# Autodesk Inventor assembly: Голень в сборе_MIR
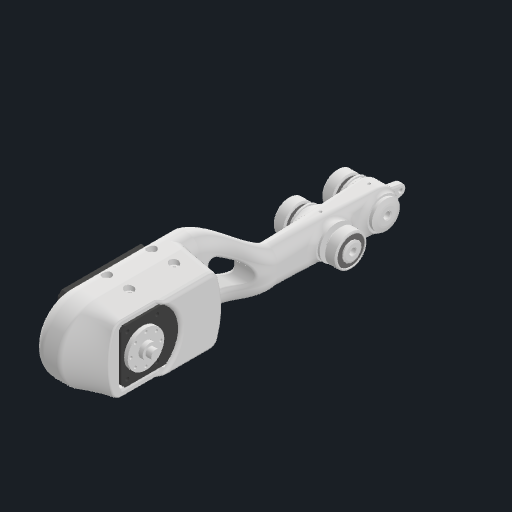
[picture p0: Inventor's stored thumbnail of the model, 512x512]
Saved by Autodesk Inventor 2025 (Build 290162010, 162A)
## iProperties
Created: 2024-12-05
Part Number: Голень в сборе_MIR
Document SubType Name: Assembly
Designer: Edward_Higgins
Author: Edward_Higgins
## Documents named in this file (8)
- D:\Users\Edward_Higgins\Desktop\ZAVOD\Робот Сколково\Голень в сборе_MIR.iam
- D:\Users\Edward_Higgins\Desktop\ZAVOD\Робот Сколково\DYNAMIXEL XM430-W350.ipt
- D:\Users\Edward_Higgins\Desktop\ZAVOD\Робот Сколково\Нога_MIR.ipt
- D:\Users\Edward_Higgins\Desktop\ZAVOD\Робот Сколково\Подшипник.ipt
- D:\Users\Edward_Higgins\Desktop\ZAVOD\Робот Сколково\Ось двусторонняя.ipt
- D:\Users\Edward_Higgins\Desktop\ZAVOD\Робот Сколково\Шайба.ipt
- D:\Users\Edward_Higgins\Desktop\ZAVOD\Робот Сколково\Стопорная шайба.ipt
- D:\Users\Edward_Higgins\Desktop\ZAVOD\Робот Сколково\Ось односторонняя.ipt
## Components (13 placed, 7 different names)
1. DYNAMIXEL XM430-W350:1 — Совмещение:4, Совмещение:8, Совмещение:7
2. Нога_MIR:1 — Совмещение:8, Совмещение:7, Совмещение:6, Совмещение:17, Совмещение:21, Совмещение:20, Совмещение:31, Совмещение:30, Совмещение:26
3. Подшипник:1 — Совмещение:19, Совмещение:9, Совмещение:15
4. Подшипник:2 — Совмещение:18, Совмещение:10, Совмещение:22, Совмещение:16
5. Ось двусторонняя:1 — Совмещение:19, Совмещение:18, Совмещение:17, Совмещение:10, Совмещение:9, Совмещение:11, Совмещение:12, Совмещение:14, Совмещение:13
6. Шайба:1 — Совмещение:21, Совмещение:11
7. Шайба:2 — Совмещение:22, Совмещение:20, Совмещение:12
8. Стопорная шайба:1 — Совмещение:15, Совмещение:14
9. Стопорная шайба:2 — Совмещение:16, Совмещение:13
10. Подшипник:3 — Совмещение:24, Совмещение:23, Совмещение:28, Совмещение:25
11. Стопорная шайба:3 — Совмещение:24, Совмещение:23
12. Шайба:3 — Совмещение:31, Совмещение:29
13. Ось односторонняя:1 — Совмещение:30, Совмещение:26, Совмещение:29, Совмещение:28, Совмещение:25
## Relationships (26: Mate 25, Flush 1)
- Совмещение:4 [Flush]: DYNAMIXEL XM430-W350:1
- Совмещение:8 [Mate]: DYNAMIXEL XM430-W350:1 ↔ Нога_MIR:1
- Совмещение:7 [Mate] (0.25 mm): DYNAMIXEL XM430-W350:1 ↔ Нога_MIR:1
- Совмещение:6 [Mate]: Нога_MIR:1
- Совмещение:19 [Mate]: Подшипник:1 ↔ Ось двусторонняя:1
- Совмещение:18 [Mate]: Подшипник:2 ↔ Ось двусторонняя:1
- Совмещение:17 [Mate]: Нога_MIR:1 ↔ Ось двусторонняя:1
- Совмещение:10 [Mate]: Подшипник:2 ↔ Ось двусторонняя:1
- Совмещение:9 [Mate]: Подшипник:1 ↔ Ось двусторонняя:1
- Совмещение:21 [Mate]: Нога_MIR:1 ↔ Шайба:1
- Совмещение:11 [Mate]: Ось двусторонняя:1 ↔ Шайба:1
- Совмещение:22 [Mate] (2 mm): Подшипник:2 ↔ Шайба:2
- Совмещение:20 [Mate]: Нога_MIR:1 ↔ Шайба:2
- Совмещение:12 [Mate]: Ось двусторонняя:1 ↔ Шайба:2
- Совмещение:15 [Mate]: Подшипник:1 ↔ Стопорная шайба:1
- Совмещение:14 [Mate]: Ось двусторонняя:1 ↔ Стопорная шайба:1
- Совмещение:16 [Mate]: Подшипник:2 ↔ Стопорная шайба:2
- Совмещение:13 [Mate]: Ось двусторонняя:1 ↔ Стопорная шайба:2
- Совмещение:24 [Mate]: Подшипник:3 ↔ Стопорная шайба:3
- Совмещение:23 [Mate]: Подшипник:3 ↔ Стопорная шайба:3
- Совмещение:31 [Mate]: Нога_MIR:1 ↔ Шайба:3
- Совмещение:30 [Mate]: Нога_MIR:1 ↔ Ось односторонняя:1
- Совмещение:26 [Mate]: Нога_MIR:1 ↔ Ось односторонняя:1
- Совмещение:29 [Mate]: Шайба:3 ↔ Ось односторонняя:1
- Совмещение:28 [Mate]: Подшипник:3 ↔ Ось односторонняя:1
- Совмещение:25 [Mate]: Подшипник:3 ↔ Ось односторонняя:1
